# Autodesk Inventor assembly: borewell jack
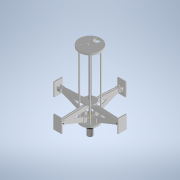
[picture p0: Inventor's stored thumbnail of the model, 180x180]
Saved by Autodesk Inventor 2021 (Build 250183000, 183)
## iProperties
Created: 2021-05-02
Part Number: borewell jack
Document SubType Name: Assembly
Designer: ASUS
Author: ASUS
## Documents named in this file (11)
- E:\borewell rescuebot\pll manipulator files\sps manipulator\borewell jack.iam
- E:\borewell rescuebot\2020 bot\Part2.ipt
- E:\borewell rescuebot\2020 bot\Part3.ipt
- E:\borewell rescuebot\2020 bot\head.ipt
- E:\borewell rescuebot\2020 bot\Part34.ipt
- E:\borewell rescuebot\2020 bot\Part37.ipt
- E:\borewell rescuebot\2020 bot\Part38.ipt
- E:\borewell rescuebot\2020 bot\Symmetry of hinge.ipt
- E:\borewell rescuebot\2020 bot\pin large.ipt
- E:\borewell rescuebot\2020 bot\endeffector motor assembly.iam
- E:\borewell rescuebot\2020 bot\lead screw for j1.ipt
## Components (37 placed, 10 different names)
1. Part2:1
2. head:1
3. Part37:1
4. Part38:1
5. Part37:2
6. Part37:3
7. Part37:4
8. endeffector motor assembly:1 [sub-assembly]
9. lead screw for j1:1
10. Symmetry of hinge:2
11. Part3:3
12. Part3:2
13. Part3:1
14. Symmetry of hinge:1
15. pin large:1
16. Part34:1
17. Symmetry of hinge:3
18. Part3:4
19. Part3:5
20. Part3:6
21. Symmetry of hinge:4
22. pin large:2
23. Part34:2
24. Symmetry of hinge:5
25. Part3:7
26. Part3:8
27. Part3:9
28. Symmetry of hinge:6
29. pin large:3
30. Part34:3
31. Symmetry of hinge:7
32. Part3:10
33. Part3:11
34. Part3:12
35. Symmetry of hinge:8
36. pin large:4
37. Part34:4
## Component patterns: (4 elements, first: Symmetry of hinge:2 + Part3:3 + Part3:2 + Part3:1 + Symmetry of hinge:1 + pin large:1 + Part34:1)
## Relationships (34: Mate 26, Flush 8)
- [Mate]: Part2:1 ↔ Part37:2
- [Flush]: Part2:1 ↔ Part37:2
- [Mate]: Part2:1 ↔ Part37:1
- [Flush]: Part2:1 ↔ Part37:1
- [Mate]: Part2:1 ↔ Part37:4
- [Flush]: Part2:1 ↔ Part37:4
- [Flush]: Part2:1 ↔ Part37:3
- [Mate]: Part2:1 ↔ Part37:3
- [Mate]: Part2:1 ↔ head:1
- [Mate]: Part3:2 ↔ Part3:1
- [Mate]: Part3:3 ↔ Part3:1
- [Mate]: Part3:2 ↔ Part3:1
- [Mate]: Part3:3 ↔ Part3:1
- [Mate]: Part3:3 ↔ Part34:1
- [Mate]: Part3:3 ↔ Part34:1
- [Mate]: Part2:1 ↔ Part3:1
- [Mate]: Part2:1 ↔ Part3:1
- [Mate]: head:1 ↔ Part3:2
- [Mate]: Part3:3 ↔ Part3:2
- [Mate]: Part2:1 ↔ Symmetry of hinge:1
- [Flush] (-2.5 mm): Part2:1 ↔ Symmetry of hinge:1
- [Mate]: Part38:1 ↔ Part37:3
- [Mate]: Part38:1 ↔ Part37:4
- [Flush]: Part38:1 ↔ Part37:4
- [Mate]: Symmetry of hinge:2 ↔ Part3:2
- [Flush] (2.5 mm): Symmetry of hinge:2 ↔ Part3:2
- [Mate]: pin large:1 ↔ Part34:1
- [Flush] (-2.5 mm): pin large:1 ↔ Part34:1
- [Mate]: Part2:1 ↔ endeffector motor assembly:1
- [Mate]: Part2:1 ↔ endeffector motor assembly:1
- [Mate]: Part2:1 ↔ endeffector motor assembly:1
- [Mate]: endeffector motor assembly:1 ↔ lead screw for j1:1
- [Mate]: Part38:1 ↔ lead screw for j1:1
- [Mate] (280 mm): head:1 ↔ Part38:1
## Named parameters: d25_d28 = 0 mm, d26_d29 = -2.5 mm, d27_d30 = 0 mm, d28_d31 = 0 mm, d29_d32 = 0 mm, d30_d33 = 0 mm, d31_d34 = 2.5 mm, d32_d35 = 0 mm, d33_d36 = -2.5 mm
